# Autodesk Inventor assembly: Wheel
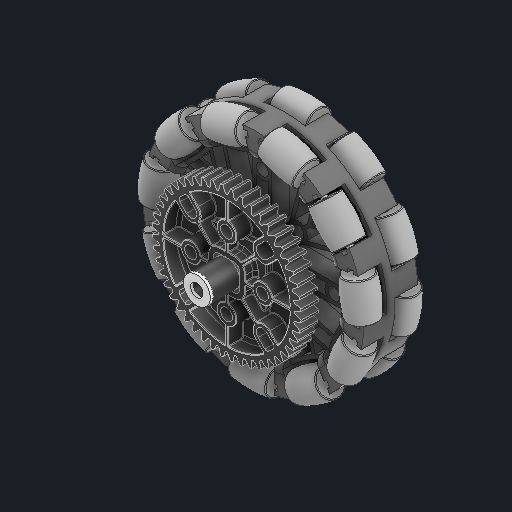
[picture p0: Inventor's stored thumbnail of the model, 512x512]
Saved by Autodesk Inventor 2025 (Build 290162000, 162)
## iProperties
Created: 2025-01-28
Part Number: Wheel
Document SubType Name: Assembly
Designer: Averey Ku
Author: Averey Ku
## Documents named in this file (11)
- D:\VEX\High Stakes\CAD\V5\Chassis\Drivebay\Wheel.iam
- D:\VEX\High Stakes\CAD\ROBOPROS-CAD-Inventor\Motion\Wheels\Omni Wheel\3.25 Omni AS, No Insert.iam
- D:\VEX\High Stakes\CAD\ROBOPROS-CAD-Inventor\Motion\Wheels\Omni Wheel.iam
- D:\VEX\High Stakes\CAD\ROBOPROS-CAD-Inventor\Modified Parts\Half Cut HS 48T Gear, No Insert.ipt
- D:\VEX\High Stakes\CAD\ROBOPROS-CAD-Inventor\Motion\Spacers\Spacer Nylon .375 OD\NSpacer .375 OD x .250.ipt
- D:\VEX\High Stakes\CAD\ROBOPROS-CAD-Inventor\Motion\Spacers\Spacer Nylon .375 OD.ipt
- D:\VEX\High Stakes\CAD\ROBOPROS-CAD-Inventor\Structure\Hardware\Nut Alu.ipt
- D:\VEX\High Stakes\CAD\ROBOPROS-CAD-Inventor\Motion\Spacers\Spacer Nylon .375 OD\NSpacer .375 OD x .375.ipt
- D:\VEX\High Stakes\CAD\ROBOPROS-CAD-Inventor\Motion\Spacers\Washer Teflon\TWasher .375 OD x .04000.ipt
- D:\VEX\High Stakes\CAD\ROBOPROS-CAD-Inventor\Motion\Spacers\Washer Teflon.ipt
- D:\VEX\High Stakes\CAD\ROBOPROS-CAD-Inventor\Structure\Hardware\Nut Nylock.ipt
## Components (9 placed, 7 different names)
1. 3.25 Omni AS, No Insert:1 [sub-assembly] — Insert:3, Mate:1, Insert:4, Insert:5, Insert:8
2. Half Cut HS 48T Gear, No Insert:1 — Insert:1, Insert:2, Mate:1, Insert:6
3. NSpacer .375 OD x .250:1 — Insert:1
4. NSpacer .375 OD x .250:2 — Insert:2, Insert:3
5. Nut Alu:1 — Insert:5
6. Nut Alu:2 — Insert:4
7. NSpacer .375 OD x .375:3 — Insert:6, Insert:7
8. TWasher .375 OD x .04000:1 — Insert:7
9. Nut Nylock:1 — Insert:8
## Relationships (9: Insert 8, Mate 1)
- Insert:1: Half Cut HS 48T Gear, No Insert:1 ↔ NSpacer .375 OD x .250:1
- Insert:2: Half Cut HS 48T Gear, No Insert:1 ↔ NSpacer .375 OD x .250:2
- Insert:3: 3.25 Omni AS, No Insert:1 ↔ NSpacer .375 OD x .250:2
- Mate:1: 3.25 Omni AS, No Insert:1 ↔ Half Cut HS 48T Gear, No Insert:1
- Insert:4: 3.25 Omni AS, No Insert:1 ↔ Nut Alu:2
- Insert:5: 3.25 Omni AS, No Insert:1 ↔ Nut Alu:1
- Insert:6: Half Cut HS 48T Gear, No Insert:1 ↔ NSpacer .375 OD x .375:3
- Insert:7: NSpacer .375 OD x .375:3 ↔ TWasher .375 OD x .04000:1
- Insert:8: 3.25 Omni AS, No Insert:1 ↔ Nut Nylock:1
